# Autodesk Inventor assembly: Right Back Drive Wheel Assembly
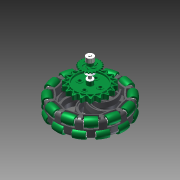
[picture p0: Inventor's stored thumbnail of the model, 180x180]
Saved by Autodesk Inventor 2012 (Build 160160000, 160)
## iProperties
Created: 2011-09-10
Part Number: Right Back Drive Wheel Assembly
Document SubType Name: Assembly
Designer: Wade
Author: Wade
## Documents named in this file (9)
- C:\Users\Wade\Documents\1103 Robot - CAD Assembly\Right Back Drive Wheel Assembly.iam
- C:\Users\Wade\Documents\1103 Robot - CAD Assembly\18 Tooth HS Sprocket.ipt
- C:\Users\Wade\Documents\24C VEX CAD Files\Wheels\4'' Omni-Directional Wheel.iam
- C:\Users\Wade\Documents\24C VEX CAD Files\Washers & Spacers\Spacer (Nylon), 0.500''.ipt
- C:\Users\Wade\Documents\24C VEX CAD Files\Washers & Spacers\Washer, Delrin.ipt
- C:\Users\Wade\Documents\24C VEX CAD Files\Other Parts\Shaft Collar (with Set Screw Installed).ipt
- C:\Users\Wade\Documents\24C VEX CAD Files\Drive Shafts\Drive Shaft (Square Bar) 3.625''.ipt
- C:\Users\Wade\Documents\24C VEX CAD Files\Washers & Spacers\Spacer (Nylon), 0.125''.ipt
- C:\Users\Wade\Documents\24C VEX CAD Files\Gears & Pulleys\24-Tooth Sprocket.ipt
## Components (9 placed, 8 different names)
1. 18 Tooth HS Sprocket:1 — Flush:1, Flush:3, Mate:6, Mate:10, Mate:11, Mate:14, Mate:16
2. 4'' Omni-Directional Wheel:1 [sub-assembly] — Mate:1, Flush:1, Mate:3, Flush:2, Flush:3, Mate:8, Mate:9
3. Spacer (Nylon), 0.500'':1 — Mate:1, Mate:9
4. Washer, Delrin:1 — Mate:6, Mate:11, Mate:15
5. Shaft Collar (with Set Screw Installed):1 — Mate:3, Flush:2, Mate:8, Mate:10
6. Drive Shaft (Square Bar) 3.625'':1 — Flush:5, Flush:6
7. Spacer (Nylon), 0.125'':1 — Mate:14, Mate:15, Mate:17
8. 24-Tooth Sprocket:1 — Mate:16, Flush:5, Mate:17, Mate:18, Mate:19
9. Shaft Collar (with Set Screw Installed):2 — Mate:18, Mate:19, Flush:6
## Relationships (21: Mate 15, Flush 6)
- Mate:1: 4'' Omni-Directional Wheel:1 ↔ Spacer (Nylon), 0.500'':1
- Flush:1: 18 Tooth HS Sprocket:1 ↔ 4'' Omni-Directional Wheel:1
- Mate:3: 4'' Omni-Directional Wheel:1 ↔ Shaft Collar (with Set Screw Installed):1
- Flush:2: 4'' Omni-Directional Wheel:1 ↔ Shaft Collar (with Set Screw Installed):1
- Flush:3: 18 Tooth HS Sprocket:1 ↔ 4'' Omni-Directional Wheel:1
- Mate:6: 18 Tooth HS Sprocket:1 ↔ Washer, Delrin:1
- Mate:8: 4'' Omni-Directional Wheel:1 ↔ Shaft Collar (with Set Screw Installed):1
- Mate:9: 4'' Omni-Directional Wheel:1 ↔ Spacer (Nylon), 0.500'':1
- Mate:10: 18 Tooth HS Sprocket:1 ↔ Shaft Collar (with Set Screw Installed):1
- Mate:11: 18 Tooth HS Sprocket:1 ↔ Washer, Delrin:1
- [Mate]: 18 Tooth HS Sprocket:1 ↔ Drive Shaft (Square Bar) 3.625'':1
- [Mate]: 18 Tooth HS Sprocket:1 ↔ Drive Shaft (Square Bar) 3.625'':1
- [Flush] (-6.35 mm): Spacer (Nylon), 0.500'':1 ↔ Drive Shaft (Square Bar) 3.625'':1
- Mate:14: 18 Tooth HS Sprocket:1 ↔ Spacer (Nylon), 0.125'':1
- Mate:15 (7.5184 mm): Washer, Delrin:1 ↔ Spacer (Nylon), 0.125'':1
- Mate:16: 18 Tooth HS Sprocket:1 ↔ 24-Tooth Sprocket:1
- Flush:5: Drive Shaft (Square Bar) 3.625'':1 ↔ 24-Tooth Sprocket:1
- Mate:17: Spacer (Nylon), 0.125'':1 ↔ 24-Tooth Sprocket:1
- Mate:18: 24-Tooth Sprocket:1 ↔ Shaft Collar (with Set Screw Installed):2
- Mate:19: 24-Tooth Sprocket:1 ↔ Shaft Collar (with Set Screw Installed):2
- Flush:6: Drive Shaft (Square Bar) 3.625'':1 ↔ Shaft Collar (with Set Screw Installed):2
